# Autodesk Inventor assembly: Assembly_Cube_Kinematic_Mirrormount_Astromedia_30x40x1_90_PRO_magnetic
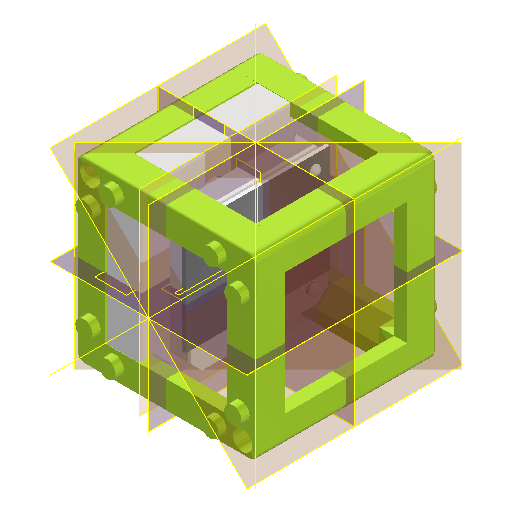
[picture p0: Inventor's stored thumbnail of the model, 512x512]
Saved by Autodesk Inventor 2022 (Build 260153000, 153)
## iProperties
Created: 2021-11-15
Part Number: Assembly_Cube_Kinematic_Mirrormount_Astromedia_30x40x1_90_PRO_magnetic
Document SubType Name: Assembly
Designer: diederichbenedict
Author: diederichbenedict
## Documents named in this file (8)
- C:\Users\diederichbenedict\Dropbox\Dokumente\Promotion\PROJECTS\openUC2-CAD\INVENTOR\Assembly_Cube_Kinematic_Mirrormount_Astromedia_30x40x1_90_PRO_magnetic.iam
- C:\Users\diederichbenedict\Dropbox\Dokumente\Promotion\PROJECTS\openUC2-CAD\INVENTOR\Assembly_Cube_empty_IM_v3.iam
- C:\Users\diederichbenedict\Dropbox\Dokumente\Promotion\PROJECTS\openUC2-CAD\INVENTOR\20_Cube_Insert_Kinematic_Astromedia_30x40x1_45_pro_magnetic.ipt
- C:\Users\diederichbenedict\Dropbox\Dokumente\Promotion\PROJECTS\openUC2-CAD\INVENTOR\20_Cube_Insert_Kinematic_Mirror_90_pro_magnetic.ipt
- C:\Users\diederichbenedict\Dropbox\Dokumente\Promotion\PROJECTS\openUC2-CAD\INVENTOR\00_Screw_Ball_Spring_Head_M3x30mm.ipt
- C:\Users\diederichbenedict\Dropbox\Dokumente\Promotion\PROJECTS\openUC2-CAD\INVENTOR\00_Threaded_Screw_Insert_M3.ipt
- C:\Users\diederichbenedict\Dropbox\Dokumente\Promotion\PROJECTS\openUC2-CAD\INVENTOR\00_NeoDymMagnet_8x3mm.ipt
- C:\Users\diederichbenedict\Dropbox\Dokumente\Promotion\PROJECTS\openUC2-CAD\INVENTOR\00_Astromedia_FronSurfaceMirror_40x30mmx1mm.ipt
## Components (14 placed, 7 different names)
1. Assembly_Cube_empty_IM_v3:1 [sub-assembly] — Angle:2, Mate:5
2. 20_Cube_Insert_Kinematic_Mirror_90_pro_magnetic:1 — Angle:2, Mate:5, Flush:1, Flush:2, Einfügen:1, Einfügen:2, Einfügen:3, Einfügen:4, Einfügen:5, Einfügen:6
3. 20_Cube_Insert_Kinematic_Astromedia_30x40x1_45_pro_magnetic:1 — Flush:1, Flush:2, Einfügen:7, Einfügen:8, Einfügen:9, Einfügen:10, Passend:6
4. 00_Screw_Ball_Spring_Head_M3x30mm:1 — Einfügen:5
5. 00_Threaded_Screw_Insert_M3:1 — Einfügen:3
6. 00_Screw_Ball_Spring_Head_M3x30mm:2 — Einfügen:6
7. 00_Threaded_Screw_Insert_M3:2 — Einfügen:2
8. 00_Screw_Ball_Spring_Head_M3x30mm:3 — Einfügen:4
9. 00_Threaded_Screw_Insert_M3:3 — Einfügen:1
10. 00_NeoDymMagnet_8x3mm:1 — Einfügen:7
11. 00_NeoDymMagnet_8x3mm:2 — Einfügen:8
12. 00_NeoDymMagnet_8x3mm:3 — Einfügen:10
13. 00_NeoDymMagnet_8x3mm:4 — Einfügen:9
14. 00_Astromedia_FronSurfaceMirror_40x30mmx1mm:1 — Passend:6
## Relationships (15: Insert 10, Mate 2, Flush 2, Angle 1)
- Angle:2 (0 deg): Assembly_Cube_empty_IM_v3:1 ↔ 20_Cube_Insert_Kinematic_Mirror_90_pro_magnetic:1
- Mate:5: Assembly_Cube_empty_IM_v3:1 ↔ 20_Cube_Insert_Kinematic_Mirror_90_pro_magnetic:1
- Flush:1: 20_Cube_Insert_Kinematic_Mirror_90_pro_magnetic:1 ↔ 20_Cube_Insert_Kinematic_Astromedia_30x40x1_45_pro_magnetic:1
- Flush:2 (2 mm): 20_Cube_Insert_Kinematic_Mirror_90_pro_magnetic:1 ↔ 20_Cube_Insert_Kinematic_Astromedia_30x40x1_45_pro_magnetic:1
- Einfügen:1 [Insert]: 20_Cube_Insert_Kinematic_Mirror_90_pro_magnetic:1 ↔ 00_Threaded_Screw_Insert_M3:3
- Einfügen:2 [Insert]: 20_Cube_Insert_Kinematic_Mirror_90_pro_magnetic:1 ↔ 00_Threaded_Screw_Insert_M3:2
- Einfügen:3 [Insert]: 20_Cube_Insert_Kinematic_Mirror_90_pro_magnetic:1 ↔ 00_Threaded_Screw_Insert_M3:1
- Einfügen:4 [Insert] (-10 mm): 20_Cube_Insert_Kinematic_Mirror_90_pro_magnetic:1 ↔ 00_Screw_Ball_Spring_Head_M3x30mm:3
- Einfügen:5 [Insert] (-10 mm): 20_Cube_Insert_Kinematic_Mirror_90_pro_magnetic:1 ↔ 00_Screw_Ball_Spring_Head_M3x30mm:1
- Einfügen:6 [Insert] (-10 mm): 20_Cube_Insert_Kinematic_Mirror_90_pro_magnetic:1 ↔ 00_Screw_Ball_Spring_Head_M3x30mm:2
- Einfügen:7 [Insert]: 20_Cube_Insert_Kinematic_Astromedia_30x40x1_45_pro_magnetic:1 ↔ 00_NeoDymMagnet_8x3mm:1
- Einfügen:8 [Insert]: 20_Cube_Insert_Kinematic_Astromedia_30x40x1_45_pro_magnetic:1 ↔ 00_NeoDymMagnet_8x3mm:2
- Einfügen:9 [Insert]: 20_Cube_Insert_Kinematic_Astromedia_30x40x1_45_pro_magnetic:1 ↔ 00_NeoDymMagnet_8x3mm:4
- Einfügen:10 [Insert]: 20_Cube_Insert_Kinematic_Astromedia_30x40x1_45_pro_magnetic:1 ↔ 00_NeoDymMagnet_8x3mm:3
- Passend:6 [Mate]: 20_Cube_Insert_Kinematic_Astromedia_30x40x1_45_pro_magnetic:1 ↔ 00_Astromedia_FronSurfaceMirror_40x30mmx1mm:1
